# Autodesk Inventor assembly: Cortemadera
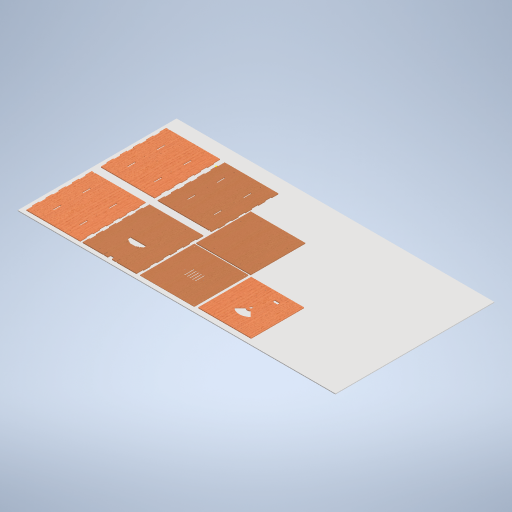
[picture p0: Inventor's stored thumbnail of the model, 512x512]
Saved by Autodesk Inventor 2024 (Build 280153000, 153)
## iProperties
Created: 2024-07-25
Part Number: Cortemadera
Document SubType Name: Assembly
Designer: sergi
Author: sergi
## Documents named in this file (9)
- C:\Users\sergi\OneDrive\Escritorio\proyectos\ComederoV6\Cortemadera.iam
- C:\Users\sergi\OneDrive\Escritorio\proyectos\ComederoV6\TableroMadera.ipt
- C:\Users\sergi\OneDrive\Escritorio\proyectos\ComederoV6\Envolvente_Pared_Derecha.ipt
- C:\Users\sergi\OneDrive\Escritorio\proyectos\ComederoV6\Envolvente_Pared_Trasera.ipt
- C:\Users\sergi\OneDrive\Escritorio\proyectos\ComederoV6\Envolvente_Pared_1.ipt
- C:\Users\sergi\OneDrive\Escritorio\proyectos\ComederoV6\Envolvente_Pared_2.ipt
- C:\Users\sergi\OneDrive\Escritorio\proyectos\ComederoV6\Tapa_Inferior.ipt
- C:\Users\sergi\OneDrive\Escritorio\proyectos\ComederoV6\Tapadera.ipt
- C:\Users\sergi\OneDrive\Escritorio\proyectos\ComederoV6\Soporte_Dosificador.ipt
## Components (8 placed, 8 different names)
1. TableroMadera:1 — Coincidencia:1, Coincidencia:2, Coincidencia:3, Coincidencia:4, Coincidencia:5, Coincidencia:6, Coincidencia:7
2. Envolvente_Pared_Derecha:1 — Coincidencia:2
3. Envolvente_Pared_Trasera:1 — Coincidencia:1
4. Envolvente_Pared_1:1 — Coincidencia:4
5. Envolvente_Pared_2:1 — Coincidencia:3
6. Tapa_Inferior:1 — Coincidencia:5
7. Tapadera:1 — Coincidencia:6
8. Soporte_Dosificador:1 — Coincidencia:7
## Relationships (7: Mate 7)
- Coincidencia:1 [Mate]: TableroMadera:1 ↔ Envolvente_Pared_Trasera:1
- Coincidencia:2 [Mate]: TableroMadera:1 ↔ Envolvente_Pared_Derecha:1
- Coincidencia:3 [Mate]: TableroMadera:1 ↔ Envolvente_Pared_2:1
- Coincidencia:4 [Mate]: TableroMadera:1 ↔ Envolvente_Pared_1:1
- Coincidencia:5 [Mate]: TableroMadera:1 ↔ Tapa_Inferior:1
- Coincidencia:6 [Mate]: TableroMadera:1 ↔ Tapadera:1
- Coincidencia:7 [Mate]: TableroMadera:1 ↔ Soporte_Dosificador:1
